# Autodesk Inventor assembly: Assembly1
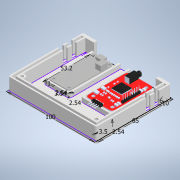
[picture p0: Inventor's stored thumbnail of the model, 180x180]
Saved by Autodesk Inventor 2020.2 (Build 242310000, 310)
## iProperties
Created: 2019-12-08
Part Number: Assembly1
Document SubType Name: Assembly
Designer: athiy
Author: athiy
## Documents named in this file (4)
- C:\Users\athiy\OneDrive\S2\01 KULIAH\SURG0094 Group Research Project\3D drawing\Assembly1.iam
- C:\Users\athiy\OneDrive\S2\01 KULIAH\SURG0094 Group Research Project\3D drawing\Part1.ipt
- C:\Users\athiy\OneDrive\S2\01 KULIAH\SURG0094 Group Research Project\3D drawing\Adafruit Feather Bluefruit 32u4 v1.ipt
- C:\Users\athiy\OneDrive\S2\01 KULIAH\SURG0094 Group Research Project\3D drawing\Voice Recognition Module.ipt
## Components (3 placed, 3 different names)
1. Part1:1 — Mate:1, Mate:2, Mate:3, Mate:4, Mate:5
2. Adafruit Feather Bluefruit 32u4 v1:1 — Mate:1, Mate:2, Mate:3
3. Voice Recognition Module:1 — Mate:4, Mate:5
## Relationships (5: Mate 5)
- Mate:1: Part1:1 ↔ Adafruit Feather Bluefruit 32u4 v1:1
- Mate:2: Part1:1 ↔ Adafruit Feather Bluefruit 32u4 v1:1
- Mate:3: Part1:1 ↔ Adafruit Feather Bluefruit 32u4 v1:1
- Mate:4: Part1:1 ↔ Voice Recognition Module:1
- Mate:5: Part1:1 ↔ Voice Recognition Module:1
